# Autodesk Inventor assembly: 155 part 2
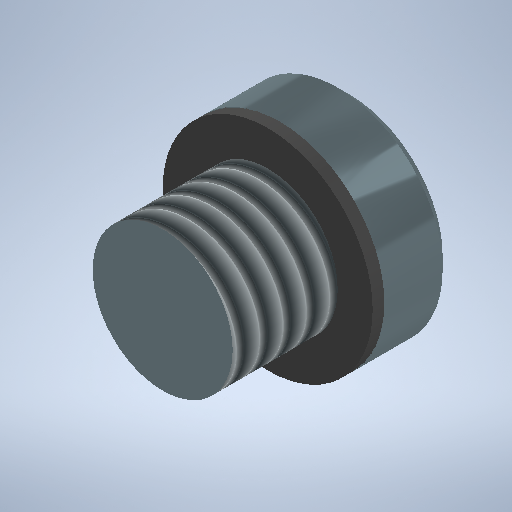
[picture p0: Inventor's stored thumbnail of the model, 512x512]
Saved by Autodesk Inventor 2025.1 (Build 291241000, 241)
## iProperties
Created: 2024-08-03
Part Number: 155 part 2
Document SubType Name: Assembly
Designer: ffogue
Author: ffogue
## Documents named in this file (3)
- C:\Projkete - Übungen\Freedom\155 part 2.iam
- C:\Projkete - Übungen\Freedom\155 part 2.ipt
- C:\Projkete - Übungen\Freedom\sicherung 155 part 2.ipt
## Components (2 placed, 2 different names)
1. 155 part 2:1 — Flush:1
2. sicherung 155 part 2:1 — Flush:1
## Relationships (1: Flush 1)
- Flush:1: 155 part 2:1 ↔ sicherung 155 part 2:1
